# Autodesk Inventor assembly: ropeDriver
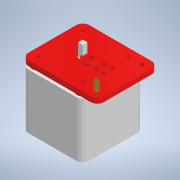
[picture p0: Inventor's stored thumbnail of the model, 180x180]
Saved by Autodesk Inventor 2020 (Build 240168000, 168)
## iProperties
Created: 2020-02-03
Part Number: ropeDriver
Document SubType Name: Assembly
Designer: Felix
Author: Felix
## Documents named in this file (5)
- C:\Users\Felix\Documents\Programmieren\ropeBot\testBotV1\ropeDriver.iam
- C:\Users\Felix\Documents\Programmieren\ropeBot\testBotV1\stepper.ipt
- C:\Users\Felix\Documents\Programmieren\ropeBot\testBotV1\housing.ipt
- C:\Users\Felix\Documents\Programmieren\ropeBot\testBotV1\brassPin.ipt
- C:\Users\Felix\Documents\Programmieren\ropeBot\testBotV1\pulley.ipt
## Components (4 placed, 4 different names)
1. stepper:1 — Flush:1
2. housing:1 — Flush:1, Mate:1, Flush:2, Flush:3
3. brassPin:1 — Mate:1, Flush:2
4. pulley:1 — Flush:3
## Relationships (4: Flush 3, Mate 1)
- Flush:1 (2 mm): stepper:1 ↔ housing:1
- Mate:1: housing:1 ↔ brassPin:1
- Flush:2: housing:1 ↔ brassPin:1
- Flush:3: housing:1 ↔ pulley:1
